# Autodesk Inventor assembly: Middle8inWheel
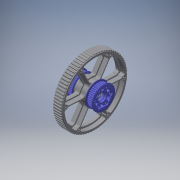
[picture p0: Inventor's stored thumbnail of the model, 180x180]
Saved by Autodesk Inventor 2016 (Build 200138000, 138)
## iProperties
Created: 2016-01-27
Part Number: Middle8inWheel
Document SubType Name: Assembly
Designer: 17swamipr
Author: 17swamipr
## Documents named in this file (3)
- C:\Users\PrashantBIA\Desktop\Robotics\Robot Assembly\Special Assemblies\Middle8inWheel.iam
- C:\Users\PrashantBIA\Desktop\Robotics\Robot Assembly\Special Assemblies\8inWheel.iam
- C:\Users\PrashantBIA\Desktop\Robotics\Robot Assembly\Drive Train\am-2234_42toothHTDpulleyHalfRev2.ipt
## Components (3 placed, 2 different names)
1. 8inWheel:1 [sub-assembly] — Mate:1, Mate:2
2. am-2234_42toothHTDpulleyHalfRev2:1 — Mate:2
3. am-2234_42toothHTDpulleyHalfRev2:2 — Mate:1
## Relationships (4: Insert 2, Mate 2)
- [Insert]: am-2234_42toothHTDpulleyHalfRev2:1 ↔ am-2234_42toothHTDpulleyHalfRev2:2
- [Insert]: am-2234_42toothHTDpulleyHalfRev2:1 ↔ am-2234_42toothHTDpulleyHalfRev2:2
- Mate:1: 8inWheel:1 ↔ am-2234_42toothHTDpulleyHalfRev2:2
- Mate:2: 8inWheel:1 ↔ am-2234_42toothHTDpulleyHalfRev2:1
